# Autodesk Inventor assembly: Door_Levered
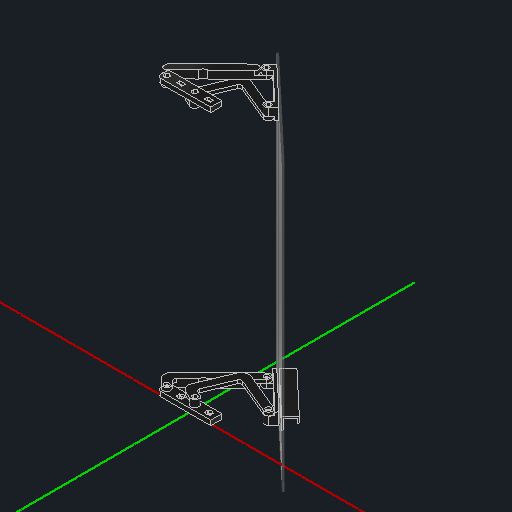
[picture p0: Inventor's stored thumbnail of the model, 512x512]
Saved by Autodesk Inventor 2022.2 (Build 262287010, 287A)
## iProperties
Created: 2022-01-24
Part Number: Door_Levered
Document SubType Name: Assembly
Designer: sleib
Author: sleib
## Documents named in this file (10)
- C:\Users\sleib\Projekte\Voron-2\CAD\Inventor\Door Levered [A].iam
- C:\Users\sleib\Projekte\Voron-2\CAD\Inventor\Door Basis.ipt
- C:\Users\sleib\Projekte\Voron-2\CAD\Inventor\Door Lever [A].ipt
- C:\Users\sleib\Projekte\Voron-2\CAD\Inventor\Door Panel [A].ipt
- C:\Users\sleib\Projekte\Voron-2\CAD\Inventor\Door Lever2 [A].ipt
- C:\Users\sleib\Projekte\Voron-2\CAD\Inventor\Door Handle.ipt
- C:\Users\sleib\Projekte\Voron-2\CAD\Inventor\Door Lever [B].ipt
- C:\Users\sleib\Projekte\Voron-2\CAD\Inventor\Door Lever2 [B].ipt
- C:\Users\sleib\Projekte\Voron-2\CAD\Inventor\Door Panel [B].ipt
- C:\Users\sleib\Projekte\Voron-2\CAD\Inventor\Panel Door.ipt
## Components (10 placed, 9 different names)
1. Door Basis:1 — Passend:4, Passend:10, Passend:12, Passend:13, Winkel:1, Fluchtend:1, Fluchtend:3, Fluchtend:4, Passend:30
2. Door Lever [A]:2 — Passend:4, Passend:12, Passend:17, Passend:18
3. Door Lever2 [A]:1 — Passend:10, Passend:13, Winkel:1, Passend:15, Passend:29
4. Door Panel [A]:1 — Passend:15, Passend:17, Passend:18, Passend:29, Fluchtend:2, Passend:31, Fluchtend:6, Symmetrie:1, Fluchtend:7, Fluchtend:1
5. Door Handle:1 — Fluchtend:2, Passend:33, Fluchtend:7
6. Door Basis:2 — Passend:21, Passend:22, Passend:23, Passend:24, Fluchtend:3, Fluchtend:4, Passend:30
7. Door Lever [B]:1 — Passend:21, Passend:24, Passend:26, Passend:28
8. Door Lever2 [B]:1 — Passend:22, Passend:23, Passend:25, Passend:27
9. Door Panel [B]:1 — Passend:25, Passend:26, Passend:27, Passend:28, Passend:32, Symmetrie:1
10. Panel Door:1 — Passend:31, Passend:32, Fluchtend:6, Passend:33
## Relationships (28: Mate 20, Flush 6, Angle 1, Symmetry 1)
- Passend:4 [Mate]: Door Basis:1 ↔ Door Lever [A]:2
- Passend:10 [Mate]: Door Basis:1 ↔ Door Lever2 [A]:1
- Passend:12 [Mate]: Door Basis:1 ↔ Door Lever [A]:2
- Passend:13 [Mate]: Door Basis:1 ↔ Door Lever2 [A]:1
- Winkel:1 [Angle] (-90 deg): Door Basis:1 ↔ Door Lever2 [A]:1
- Passend:15 [Mate]: Door Lever2 [A]:1 ↔ Door Panel [A]:1
- Passend:17 [Mate]: Door Lever [A]:2 ↔ Door Panel [A]:1
- Passend:18 [Mate]: Door Lever [A]:2 ↔ Door Panel [A]:1
- Passend:29 [Mate]: Door Lever2 [A]:1 ↔ Door Panel [A]:1
- Fluchtend:2 [Flush]: Door Panel [A]:1 ↔ Door Handle:1
- Passend:21 [Mate]: Door Basis:2 ↔ Door Lever [B]:1
- Passend:22 [Mate]: Door Basis:2 ↔ Door Lever2 [B]:1
- Passend:23 [Mate]: Door Basis:2 ↔ Door Lever2 [B]:1
- Passend:24 [Mate]: Door Basis:2 ↔ Door Lever [B]:1
- Passend:25 [Mate]: Door Lever2 [B]:1 ↔ Door Panel [B]:1
- Passend:26 [Mate]: Door Lever [B]:1 ↔ Door Panel [B]:1
- Passend:27 [Mate]: Door Lever2 [B]:1 ↔ Door Panel [B]:1
- Passend:28 [Mate]: Door Lever [B]:1 ↔ Door Panel [B]:1
- Fluchtend:3 [Flush]: Door Basis:1 ↔ Door Basis:2
- Fluchtend:4 [Flush]: Door Basis:1 ↔ Door Basis:2
- Passend:30 [Mate] (-490 mm): Door Basis:1 ↔ Door Basis:2
- Passend:31 [Mate]: Door Panel [A]:1 ↔ Panel Door:1
- Passend:32 [Mate]: Door Panel [B]:1 ↔ Panel Door:1
- Fluchtend:6 [Flush] (-13.4 mm): Door Panel [A]:1 ↔ Panel Door:1
- Symmetrie:1: Door Panel [A]:1 ↔ Door Panel [B]:1
- Passend:33 [Mate]: Door Handle:1 ↔ Panel Door:1
- Fluchtend:7 [Flush]: Door Panel [A]:1 ↔ Door Handle:1
- Fluchtend:1 [Flush] (-3 mm): Door Basis:1 ↔ Door Panel [A]:1
